# Autodesk Inventor assembly: 17HM15-0904S
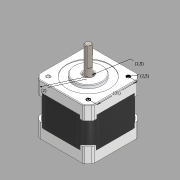
[picture p0: Inventor's stored thumbnail of the model, 180x180]
Saved by Autodesk Inventor 2022.2 (Build 262287000, 287)
## iProperties
Created: 2022-07-20
Part Number: 17HM15-0904S
Description: STEP AP214
Document SubType Name: Assembly
Designer: User
Sending System: SolidWorks 2020
Preprocessor: SwSTEP 2.0
r_shaft: 2,500 mm
x_holes: 31,000 mm
d_holes: 2,500 mm
r_flange: 2,000 mm
Title: 17HM15-0904S.STEP
Revision Number: ANY
## Documents named in this file (6)
- C:\Users\Ilewicz\Documents\Inventor\Wire Bender\NEMA17\Inventor\17HM15-0904S.iam
- C:\Users\Ilewicz\Documents\Inventor\Wire Bender\NEMA17\Inventor\nema17_bottom_40mm___ _________.ipt
- C:\Users\Ilewicz\Documents\Inventor\Wire Bender\NEMA17\Inventor\radial ball bearing_68_din_PreviewCfg.ipt
- C:\Users\Ilewicz\Documents\Inventor\Wire Bender\NEMA17\Inventor\nema17_middle_40mm___ _________.ipt
- C:\Users\Ilewicz\Documents\Inventor\Wire Bender\NEMA17\Inventor\nema17_top_40mm___ _________.ipt
- C:\Users\Ilewicz\Documents\Inventor\Wire Bender\NEMA17\Inventor\nema17_shaft_40mm___ _________.ipt
## Components (6 placed, 6 different names)
1. nema17_bottom_40mm___ __________1
2. radial ball bearing_68_din_PreviewCfg_2
3. nema17_middle_40mm___ __________3
4. nema17_top_40mm___ __________4
5. radial ball bearing_68_din_PreviewCfg_5
6. nema17_shaft_40mm___ __________6
## Named parameters: r_shaft = 2.5 mm, x_holes = 31 mm, d_holes = 2.5 mm, r_flange = 2 mm
